# Autodesk Inventor assembly: podstawa
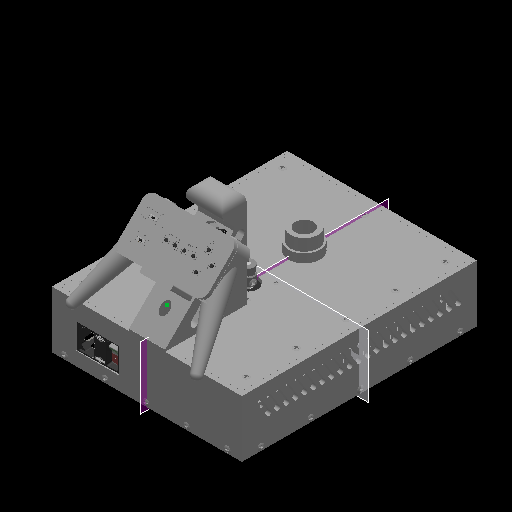
[picture p0: Inventor's stored thumbnail of the model, 512x512]
Saved by Autodesk Inventor 2024.4 (Build 284460000, 460)
## iProperties
Created: 2025-10-10
Part Number: podstawa
Document SubType Name: Assembly
Designer: User
Mass: 1308.73 g
Surface Area: 5886.67 cm^2
Volume: 1308.73 cm^3
Density: 1 g/cm^3
Author: User
## Documents named in this file (26)
- C:\Users\Duszy\Desktop\Projekty\Dummy\Dummy_v2\Model\Model\podstawa\podstawa.iam
- C:\Users\Duszy\Desktop\Projekty\Dummy\Dummy_v2\Model\Model\podstawa\podstawa_baza.ipt
- C:\Users\Duszy\Desktop\Projekty\Dummy\Dummy_v2\Model\Model\podstawa\podstawa_sciana_bok.ipt
- C:\Users\Duszy\Desktop\Projekty\Dummy\Dummy_v2\Model\Model\modele_gotowe\nema-17-stepper-motors-coaxial-60-48-39-23mm-1.snapshot.3\NEMA 17 Stepper Motor 48mm-NEMA 17 Stepper Motor 48mm.ipt
- C:\Users\Duszy\Downloads\power-supply_40a_200w-1.snapshot.1\POWER SUPPLY_40A_200W.ipt
- C:\Users\Duszy\Desktop\Projekty\Dummy\Dummy_v2\Model\Model\podstawa\podstawa_sciana_front.ipt
- C:\Users\Duszy\Desktop\Projekty\Dummy\Dummy_v2\Model\Model\podstawa\podstawa_sciana_tyl.ipt
- C:\Users\Duszy\Desktop\Projekty\Dummy\Dummy_v2\Model\Model\podstawa\podstawa_gora.ipt
- C:\Users\Duszy\Desktop\Projekty\Dummy\Dummy_v2\Model\Model\podstawa\20_zb_wal.ipt
- C:\Users\Duszy\Desktop\Projekty\Dummy\Dummy_v2\Model\Model\podstawa\94459A774_Heat-Set Inserts for Plastic.ipt
- C:\Users\Duszy\Desktop\Projekty\Dummy\Dummy_v2\Model\Model\modele_gotowe\Modele_elementów\90258A218_Phillips Oval Head Screws.ipt
- C:\Users\Duszy\Desktop\Projekty\Dummy\Dummy_v2\Model\Model\podstawa\90258A189_Phillips Oval Head Screws.ipt
- C:\Users\Duszy\Desktop\Projekty\Dummy\Dummy_v2\Model\Model\podstawa\94459A774_Heat-Set Inserts for Plastic_MIR.ipt
- C:\Users\Duszy\Desktop\Projekty\Dummy\Dummy_v2\Model\Model\modele_gotowe\Modele_elementów\90258A218_Phillips Oval Head Screws_MIR.ipt
- C:\Users\Duszy\Desktop\Projekty\Dummy\Dummy_v2\Model\Model\modele_gotowe\Modele_elementów\90258A218_Phillips Oval Head Screws_MIR1.ipt
- C:\Users\Duszy\Desktop\Projekty\Dummy\Dummy_v2\Model\Model\podstawa\94459A774_Heat-Set Inserts for Plastic_MIR1.ipt
- C:\Users\Duszy\Desktop\Projekty\Dummy\Dummy_v2\Model\Model\modele_gotowe\Modele_elementów\5428N12_IEC Connector with Power Switch.ipt
- C:\Users\Duszy\Desktop\Projekty\Dummy\Dummy_v2\Model\Model\podstawa\USB.ipt
- C:\Users\Duszy\Desktop\Projekty\Dummy\Dummy_v2\Model\Model\podstawa\podstawka.ipt
- C:\Users\Duszy\Desktop\Projekty\Dummy\Dummy_v2\Model\Model\podstawa\kontroler_bottom.ipt
- C:\Users\Duszy\Desktop\Projekty\Dummy\Dummy_v2\Model\Model\podstawa\kontroler_top.ipt
- C:\Users\Duszy\Desktop\Projekty\Dummy\Dummy_v2\Model\Model\podstawa\Micro_Button_6x6.ipt
- C:\Users\Duszy\Desktop\Projekty\Dummy\Dummy_v2\Model\Model\podstawa\SPDT slide switch SS12D00.ipt
- C:\Users\Duszy\Desktop\Projekty\Dummy\Dummy_v2\Model\Model\podstawa\ESP32 wroom 32 v9.ipt
- C:\Users\Duszy\Desktop\Projekty\Dummy\Dummy_v2\Model\Model\podstawa\skrzynka_na_elektronike.ipt
- C:\Users\Duszy\Desktop\Projekty\Dummy\Dummy_v2\PCB\main_board\main.iam
## Components (100 placed, 25 different names)
1. podstawa_baza:1 — Obrotowe:2, Obrotowe:3, Obrotowe:4, Obrotowe:5, Obrotowe:7, Obrotowe:12, Obrotowe:15, Sztywne:1, Obrotowe:28, Obrotowe:29
2. podstawa_sciana_bok:1 — Obrotowe:7, Obrotowe:20
3. podstawa_sciana_bok:2 — Sztywne:1, Obrotowe:16, Równoległe:2
4. NEMA 17 Stepper Motor 48mm-NEMA 17 Stepper Motor 48mm:1 — Obrotowe:2, Obrotowe:6, Obrotowe:8
5. POWER SUPPLY_40A_200W:1 — Obrotowe:3
6. podstawa_sciana_front:1 — Obrotowe:4
7. podstawa_sciana_tyl:1 — Obrotowe:5, Obrotowe:19, Równoległe:1, Obrotowe:22
8. podstawa_gora:1 — Obrotowe:6, Obrotowe:21, Sztywne:3, Obrotowe:24
9. 20_zb_wal:1 — Obrotowe:8, Sztywne:2
10. 94459A774_Heat-Set Inserts for Plastic_MIR:1
11. 90258A218_Phillips Oval Head Screws_MIR:1
12. 94459A774_Heat-Set Inserts for Plastic_MIR:2
13. 90258A218_Phillips Oval Head Screws_MIR:2
14. 94459A774_Heat-Set Inserts for Plastic_MIR:3
15. 90258A218_Phillips Oval Head Screws_MIR:3
16. 94459A774_Heat-Set Inserts for Plastic_MIR:4
17. 90258A218_Phillips Oval Head Screws_MIR:4
18. 94459A774_Heat-Set Inserts for Plastic_MIR:5
19. 90258A218_Phillips Oval Head Screws_MIR:5
20. 90258A218_Phillips Oval Head Screws_MIR1:1
21. 94459A774_Heat-Set Inserts for Plastic_MIR1:1
22. 90258A218_Phillips Oval Head Screws_MIR1:2
23. 94459A774_Heat-Set Inserts for Plastic_MIR1:2
24. 90258A218_Phillips Oval Head Screws_MIR1:3
25. 94459A774_Heat-Set Inserts for Plastic_MIR1:3
26. 90258A218_Phillips Oval Head Screws_MIR1:4
27. 94459A774_Heat-Set Inserts for Plastic_MIR1:4
28. 90258A218_Phillips Oval Head Screws_MIR1:5
29. 94459A774_Heat-Set Inserts for Plastic_MIR1:5
30. 5428N12_IEC Connector with Power Switch:1 — Obrotowe:22
31. 94459A774_Heat-Set Inserts for Plastic_MIR:6 — Sztywne:2, Obrotowe:23
32. 90258A218_Phillips Oval Head Screws_MIR:6 — Obrotowe:23
33. USB:1 — Sztywne:3
34. podstawka:1 — Obrotowe:24, Obrotowe:25
35. kontroler_bottom:1 — Obrotowe:25, Sztywne:4, Obrotowe:27
36. kontroler_top:1 — Sztywne:4, Obrotowe:26, Sztywne:5, Sztywne:6, Sztywne:7, Sztywne:8, Sztywne:9, Sztywne:10
37. Micro_Button_6x6:5 — Sztywne:6
38. Micro_Button_6x6:6 — Sztywne:8
39. Micro_Button_6x6:7 — Sztywne:7
40. ESP32 wroom 32 v9:1 — Obrotowe:27
41. skrzynka_na_elektronike:1 — Obrotowe:28
42. main:1 [sub-assembly] — Obrotowe:29
43. 94459A774_Heat-Set Inserts for Plastic:3 — Obrotowe:11, Obrotowe:12
44. 90258A218_Phillips Oval Head Screws:1 — Obrotowe:11
45. 94459A774_Heat-Set Inserts for Plastic:6
46. 90258A218_Phillips Oval Head Screws:4
47. 94459A774_Heat-Set Inserts for Plastic:7
48. 90258A218_Phillips Oval Head Screws:5
49. 94459A774_Heat-Set Inserts for Plastic:8
50. 90258A218_Phillips Oval Head Screws:6
51. 94459A774_Heat-Set Inserts for Plastic:9
52. 90258A218_Phillips Oval Head Screws:7
53. 90258A218_Phillips Oval Head Screws:3
54. 94459A774_Heat-Set Inserts for Plastic:5 — Obrotowe:15
55. 90258A218_Phillips Oval Head Screws:8
56. 94459A774_Heat-Set Inserts for Plastic:10
57. 90258A218_Phillips Oval Head Screws:9
58. 94459A774_Heat-Set Inserts for Plastic:11
59. 90258A218_Phillips Oval Head Screws:10
60. 94459A774_Heat-Set Inserts for Plastic:12
61. 90258A218_Phillips Oval Head Screws:11
62. 94459A774_Heat-Set Inserts for Plastic:13
63. 90258A218_Phillips Oval Head Screws:2
64. 94459A774_Heat-Set Inserts for Plastic:4 — Obrotowe:16
65. 90258A218_Phillips Oval Head Screws:12
66. 94459A774_Heat-Set Inserts for Plastic:14
67. 90258A218_Phillips Oval Head Screws:13
68. 94459A774_Heat-Set Inserts for Plastic:15
69. 90258A218_Phillips Oval Head Screws:14
70. 94459A774_Heat-Set Inserts for Plastic:16
71. 90258A218_Phillips Oval Head Screws:15
72. 94459A774_Heat-Set Inserts for Plastic:17
73. 94459A774_Heat-Set Inserts for Plastic:18 — Obrotowe:19
74. 90258A218_Phillips Oval Head Screws:16
75. 94459A774_Heat-Set Inserts for Plastic:20
76. 90258A218_Phillips Oval Head Screws:18
77. 90258A218_Phillips Oval Head Screws:17
78. 94459A774_Heat-Set Inserts for Plastic:19 — Obrotowe:20
79. 90258A218_Phillips Oval Head Screws:19
80. 94459A774_Heat-Set Inserts for Plastic:21
81. 90258A218_Phillips Oval Head Screws:20
82. 94459A774_Heat-Set Inserts for Plastic:22
83. 90258A218_Phillips Oval Head Screws:21
84. 94459A774_Heat-Set Inserts for Plastic:23
85. 90258A218_Phillips Oval Head Screws:22
86. 94459A774_Heat-Set Inserts for Plastic:24
87. 90258A189_Phillips Oval Head Screws:1 — Obrotowe:21
88. 90258A189_Phillips Oval Head Screws:2
89. 90258A189_Phillips Oval Head Screws:3
90. 90258A189_Phillips Oval Head Screws:4
91. SPDT slide switch SS12D00:1 — Obrotowe:26
92. SPDT slide switch SS12D00:2
93. Micro_Button_6x6:1 — Sztywne:5
94. Micro_Button_6x6:2
95. Micro_Button_6x6:3
96. Micro_Button_6x6:4
97. 94459A774_Heat-Set Inserts for Plastic_MIR1:6 — Sztywne:9
98. 90258A218_Phillips Oval Head Screws_MIR1:6 — Sztywne:10
99. 94459A774_Heat-Set Inserts for Plastic_MIR1:7
100. 90258A218_Phillips Oval Head Screws_MIR1:7
## Component patterns: (5 elements, first: 94459A774_Heat-Set Inserts for Plastic:3 + 90258A218_Phillips Oval Head Screws:1), (5 elements, first: 90258A218_Phillips Oval Head Screws:3 + 94459A774_Heat-Set Inserts for Plastic:5), (5 elements, first: 90258A218_Phillips Oval Head Screws:2 + 94459A774_Heat-Set Inserts for Plastic:4), (2 elements, first: 94459A774_Heat-Set Inserts for Plastic:18 + 90258A218_Phillips Oval Head Screws:16), (5 elements, first: 90258A218_Phillips Oval Head Screws:17 + 94459A774_Heat-Set Inserts for Plastic:19), (4 elements, first: 90258A189_Phillips Oval Head Screws:1), (2 elements, first: SPDT slide switch SS12D00:1), (4 elements, first: Micro_Button_6x6:1), (2 elements, first: 94459A774_Heat-Set Inserts for Plastic_MIR1:6 + 90258A218_Phillips Oval Head Screws_MIR1:6)
## Relationships (38: RevoluteJoint 26, WeldJoint 10, Flush 2)
- Obrotowe:2 [RevoluteJoint] (10 mm): podstawa_baza:1 ↔ NEMA 17 Stepper Motor 48mm-NEMA 17 Stepper Motor 48mm:1
- Obrotowe:3 [RevoluteJoint] (10 mm): podstawa_baza:1 ↔ POWER SUPPLY_40A_200W:1
- Obrotowe:4 [RevoluteJoint]: podstawa_baza:1 ↔ podstawa_sciana_front:1
- Obrotowe:5 [RevoluteJoint]: podstawa_baza:1 ↔ podstawa_sciana_tyl:1
- Obrotowe:6 [RevoluteJoint] (-5.35 mm): NEMA 17 Stepper Motor 48mm-NEMA 17 Stepper Motor 48mm:1 ↔ podstawa_gora:1
- Obrotowe:7 [RevoluteJoint]: podstawa_baza:1 ↔ podstawa_sciana_bok:1
- Obrotowe:8 [RevoluteJoint]: NEMA 17 Stepper Motor 48mm-NEMA 17 Stepper Motor 48mm:1 ↔ 20_zb_wal:1
- Obrotowe:11 [RevoluteJoint] (-6 mm): 94459A774_Heat-Set Inserts for Plastic:3 ↔ 90258A218_Phillips Oval Head Screws:1
- Obrotowe:12 [RevoluteJoint]: podstawa_baza:1 ↔ 94459A774_Heat-Set Inserts for Plastic:3
- [RevoluteJoint] (-6 mm): 90258A218_Phillips Oval Head Screws:2 ↔ 94459A774_Heat-Set Inserts for Plastic:4
- [RevoluteJoint] (-6 mm): 90258A218_Phillips Oval Head Screws:3 ↔ 94459A774_Heat-Set Inserts for Plastic:5
- Obrotowe:15 [RevoluteJoint]: podstawa_baza:1 ↔ 94459A774_Heat-Set Inserts for Plastic:5
- Sztywne:1 [WeldJoint]: podstawa_baza:1 ↔ podstawa_sciana_bok:2
- Obrotowe:16 [RevoluteJoint]: podstawa_sciana_bok:2 ↔ 94459A774_Heat-Set Inserts for Plastic:4
- [RevoluteJoint] (-6 mm): 94459A774_Heat-Set Inserts for Plastic:18 ↔ 90258A218_Phillips Oval Head Screws:16
- [RevoluteJoint] (-6 mm): 90258A218_Phillips Oval Head Screws:17 ↔ 94459A774_Heat-Set Inserts for Plastic:19
- Obrotowe:19 [RevoluteJoint]: podstawa_sciana_tyl:1 ↔ 94459A774_Heat-Set Inserts for Plastic:18
- Obrotowe:20 [RevoluteJoint]: podstawa_sciana_bok:1 ↔ 94459A774_Heat-Set Inserts for Plastic:19
- Obrotowe:21 [RevoluteJoint] (20 mm): podstawa_gora:1 ↔ 90258A189_Phillips Oval Head Screws:1
- Równoległe:1 [Flush] (-130 mm): podstawa_sciana_tyl:1
- Równoległe:2 [Flush] (-105 mm): podstawa_sciana_bok:2
- Obrotowe:22 [RevoluteJoint]: podstawa_sciana_tyl:1 ↔ 5428N12_IEC Connector with Power Switch:1
- Sztywne:2 [WeldJoint] (-0.9 mm): 20_zb_wal:1 ↔ 94459A774_Heat-Set Inserts for Plastic_MIR:6
- Obrotowe:23 [RevoluteJoint] (10 mm): 94459A774_Heat-Set Inserts for Plastic_MIR:6 ↔ 90258A218_Phillips Oval Head Screws_MIR:6
- Sztywne:3 [WeldJoint] (-13.8 mm): podstawa_gora:1 ↔ USB:1
- Obrotowe:24 [RevoluteJoint]: podstawa_gora:1 ↔ podstawka:1
- Obrotowe:25 [RevoluteJoint]: podstawka:1 ↔ kontroler_bottom:1
- Sztywne:4 [WeldJoint]: kontroler_bottom:1 ↔ kontroler_top:1
- Obrotowe:26 [RevoluteJoint] (5 mm): kontroler_top:1 ↔ SPDT slide switch SS12D00:1
- Sztywne:5 [WeldJoint] (0.5 mm): kontroler_top:1 ↔ Micro_Button_6x6:1
- Sztywne:6 [WeldJoint] (0.5 mm): kontroler_top:1 ↔ Micro_Button_6x6:5
- Sztywne:7 [WeldJoint] (0.5 mm): kontroler_top:1 ↔ Micro_Button_6x6:7
- Sztywne:8 [WeldJoint] (0.5 mm): kontroler_top:1 ↔ Micro_Button_6x6:6
- Sztywne:9 [WeldJoint]: kontroler_top:1 ↔ 94459A774_Heat-Set Inserts for Plastic_MIR1:6
- Sztywne:10 [WeldJoint] (8 mm): kontroler_top:1 ↔ 90258A218_Phillips Oval Head Screws_MIR1:6
- Obrotowe:27 [RevoluteJoint] (2.5 mm): kontroler_bottom:1 ↔ ESP32 wroom 32 v9:1
- Obrotowe:28 [RevoluteJoint]: podstawa_baza:1 ↔ skrzynka_na_elektronike:1
- Obrotowe:29 [RevoluteJoint] (-10 mm): podstawa_baza:1 ↔ main:1
## Named parameters: d40_d36 = -6 mm, d41_d37 = -55.576622 deg, d42_d40_d36 = -6 mm, d43_d41_d37 = 34.423378 deg, d61_d40_d36 = -6 mm, d62_d41_d37 = -151.290468 deg, d63_d61_d40_d36 = -6 mm, d64_d62_d41_d37 = -156.808751 deg
